# Autodesk Inventor assembly: 5A.00.01.01-IB-VTP-Master-Assy-copy
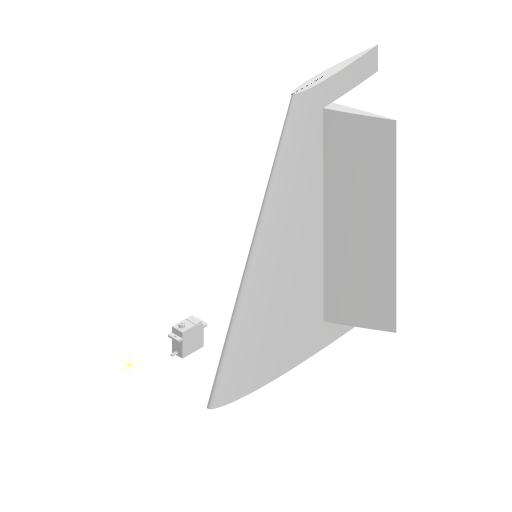
[picture p0: Inventor's stored thumbnail of the model, 512x512]
Saved by Autodesk Inventor 2024 (Build 280153000, 153)
## iProperties
Created: 2024-11-03
Part Number: 5A.00.01.01-IB-VTP-Master-Assy-copy
Document SubType Name: Assembly
Designer: inigo
Author: inigo
## Documents named in this file (5)
- C:\Users\inigo\OneDrive - University of Bristol\General - grp-Company A - AVDASI2 2024-25\CAD Files\VTP\5A.00.01.01-IB-VTP-Master-Assy-copy.iam
- C:\Users\inigo\OneDrive - University of Bristol\General - grp-Company A - AVDASI2 2024-25\CAD Files\VTP\5P.00.01.02-IB-VTP-Rudder.ipt
- C:\Users\inigo\OneDrive - University of Bristol\General - grp-Company A - AVDASI2 2024-25\CAD Files\VTP\5P.00.01.01-IB-VTP-Body.ipt
- C:\Users\inigo\OneDrive - University of Bristol\General - grp-Company A - AVDASI2 2024-25\CAD Files\VTP\5P.00.01.01-IB-VTP-Hinge-Rod.ipt
- C:\Users\inigo\OneDrive - University of Bristol\General - grp-Company A - AVDASI2 2024-25\CAD Files\VTP\EMAX-09-MD Servo.ipt
## Components (4 placed, 4 different names)
1. 5P.00.01.01-IB-VTP-Body:1 — Mate:2, Mate:3, Mate:4
2. 5P.00.01.02-IB-VTP-Rudder:1 — Mate:1, Flush:1
3. 5P.00.01.01-IB-VTP-Hinge-Rod:1 — Mate:1, Flush:1, Mate:2, Mate:3
4. EMAX-09-MD Servo:1
## Relationships (5: Mate 4, Flush 1)
- Mate:1: 5P.00.01.02-IB-VTP-Rudder:1 ↔ 5P.00.01.01-IB-VTP-Hinge-Rod:1
- Flush:1 (-10 mm): 5P.00.01.02-IB-VTP-Rudder:1 ↔ 5P.00.01.01-IB-VTP-Hinge-Rod:1
- Mate:2: 5P.00.01.01-IB-VTP-Body:1 ↔ 5P.00.01.01-IB-VTP-Hinge-Rod:1
- Mate:3 (-10 mm): 5P.00.01.01-IB-VTP-Body:1 ↔ 5P.00.01.01-IB-VTP-Hinge-Rod:1
- Mate:4: 5P.00.01.01-IB-VTP-Body:1
